# Autodesk Inventor assembly: 043.5-DQ(F,D-166-3)
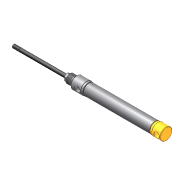
[picture p0: Inventor's stored thumbnail of the model, 180x180]
Saved by Autodesk Inventor 2012 (Build 160160000, 160)
## iProperties
Category: PARTsolutions
Created: 2013-01-20
Part Number: 043.5-DQ(F,D-166-3)
Catalog Web Link: www.cadenas.de
Description: Original Line Standard Air Cylinders -
Document SubType Name: Assembly
Designer: PARTsolutions
Mass: 32.8083 g
Surface Area: 278.831 cm^2
Volume: 32.8083 cm^3
Density: 1 g/cm^3
NB: 043.5-DQ(F,D-166-3)
NN: Original Line Standard Air Cylinders
NBSYN: $PNC.
LINA: 043.5-DQ
PSOL_MULTISOLIDPART: 0.0
PN: 043.5-DQ
PNC: 043.5-DQ(F,D-166-3)
PNA: (D-166-3)
DASH: -
BORE1: 0.75000000
BORE: 3/4" (04)
BOREPN: 04
STROKE: 3.500
STROKEALG: [0.011:50/0.001]
STROKE1: 3.500
ACTING: D
ACTINGALG: '' , 'Single Acting (SA)' , 'R' , 'Reverse Single Acting (SA)' , 'D' , 'Double Acting (SA)'
ACTINGPN: D
MNTALG: '' , 'Front Nose Mounting (SA)' , 'P' , 'Rear Pivot Mounting (SA)' , 'XP' , 'Double End or Pivot Mounting (SA)' , 'X' , 'Double End Mounting (SA)' , 'BF' , 'Front Block Mounting (SA)' , 'BR' , 'Rear Block Mounting for Vertical Positioning (SA)' , 'BFT' , 'Front Block Trunnion Mounting (SA)' , 'BRT' , 'Rear Block Trunnion Mounting (SA)'
DERALG: '' , 'N/A'
NRALG: '' , 'N/A'
BMALG: '' , 'N/A'
COALG: '' , 'N/A'
OOALG: '', 'N/A'
VO: Z
VOALG: 'Z' , 'N/A'
MALG: '', 'Without Magnet', 'M', 'With Magnet'
EEL: 0.000
EEMAX: 46.5000
EEALG: '', 'Without Extra Extension', 'EE', 'With Extra Extension'
EELALG: 0
EEPN1: 0.000
KALG: '' , 'N/A'
Q: Q
QALG: '' , 'Standard Port' , 'Q' , 'Side Port'
QPN: Q
YALG: '' , 'N/A'
FALG: '', 'Non-Coated (Standard)', 'F', 'Molycoated'
TALG: '' , 'Standard -20° to 200°F (-29° to 95°C)' , 'N' , 'Low Temperature' , 'V' , 'High Temperature'
BALG: '', 'W/out Bumpers' , 'B' , 'W/ Bumpers'
HALG: '', 'N/A'
SERALG: '' , 'Without Spring Extend/Return' , 'JS' , 'With Spring Return' , 'JR' , 'With Spring Extend'
SR: C
SRALG: 'C' , 'Standard Blackened Carbon Steel' , 'SR' , 'Stainless Steel [SR]'
SRCON: 1
WALG: '' , 'Without Wiper' , 'W' , 'With Wiper'
EALG: '' , 'Standard Seals/Lube' , 'E' , 'Non-Lube Seals/Lube'
HLALG: '' , 'Without Low Pressure Hydraulic' , 'HL' , 'With Low Pressure Hydraulic'
STALG: '' , 'N/A'
STPT1ALG: '' , 'N/A'
STPT2ALG: '' , 'N/A'
STPT3ALG: '' , 'N/A'
STPT4ALG: '' , 'N/A'
MBALG: '' , 'Without Mounting Bracket' , 'F,D-129' , 'D-129 (front)'
MBPNALL: D-129
PBALG: '' , 'N/A'
PRC: F,D-166-3
PRCALG: '' , 'W/out Pivot Rod Clevis' , 'F,D-166-3' , 'D-166-3 (front)'
PRCPN: (F,D-166-3)
PRCPNALL: D-166-3
TBALG: '' , 'N/A'
MNALG: '' , 'N/A'
TLEN: 4.7565
FRAC: 16.4700
RGDACCON: R
RHCON1: P
RHCONON: 1
FNUTCON: 1
RNUTCON: 0
FNUTPN: D-9
FNUTTRANS: 0.0000
RNUTTRANS: 0.0000
VHOLECON: 0
A1: 1.5940
A1N: 0.8750
A1P: 1.5940
A1B: 1.5940
A4: 0.2525
A4N: 0.3130
A4P: 0.2525
A5: 0.0300
A1H: 0.531
A1NH: 0.5310
A1PH: 1.5940
A1BH: 1.0940
A1SH: 1.2190
A2H: 0.2190
A2NH: 0.2190
LENGTH: 2.9700
LENGTH1: 2.9700
LENGTH2: 3.0300
MUL: 3.5000
MUL11: 3.5000
MUL22: 9.415
MUL33: 5.9150
MUL2: 3.5000
MUL211: 3.5000
MUL222: 2.6900
MUL233: 1.6900
SSS: 7.0000
RGLEN: 1.3715
RHLEN: 0.3420
SSS1: 4.0000
A13: 1.3120
DIF: 0.0000
G5: 0.6250
ON: 0
SSADD: 0.0000
BADD: 0.0000
MADD: 0.0000
NVADD: 0.0000
TRACKL: 4.4665
TRACKCON: D-74168
TRIMCON: 0
TRIMCON1: 0
FSPACE: 0.7247
SPACE: 0.0804
TEXT: 0.1406
S1: 1.0000
D1: 0.8325
D1N: 0.8050
D1B: 0.8625
D1P: 0.8325
FA: 0.940
RA: 0.9400
PPATH: standard_air_cylinder_asmtpl.prj
MATALGHTML: <b>Standard Original Line:</b><dl><dt>Rod:</dt><dd>- Stainless Steel</dd><dd>&nbsp;&nbsp;(5/16 ? 9/16 Bores)</dd><dd>- High Strength Carbon Steel</dd><dd>&nbsp;&nbsp;(3/4 ? 3 Bore)</dd><dd>- Stainless Steel</dd><dd>&nbsp;&nbsp;(?X? style DXP/DX/DXDE?)</dd><dt>Bearings:</dt><dd>- Sintered Bronze</dd><dt>Body:</dt><dd>- 304 Stainless Steel</dd><dt>End Caps:</dt><dd>- Aluminum</dd><dt>Seals:</dt><dd>- Buna N</dd></dl>
ASSCFGPRA: 04D
PRCPNA: (D-166-3)
ASSOPTACC: STPT4
A: 6.91
HADD: 0.0000
WFL: 0.250
QADD: 0.440
QADD1: 0.440
TEST: 3.0000
STDNUTF: 1
STDNUTR: 0
KT: DUMMY
CreationOption_UseAsmMates: false
SUPPLIER: Bimba
ARTICLENO: 043.5-DQ(F,D-166-3)
BOMINFO: 043.5-DQ
CREATOR: CADENAS GmbH
PSOL_IDENT_0: {\\10.0.0.242\data_v9\23d-libs\bimba\bimba\bimba_imperial\bimba_full_line\original_line_cylinders\st
PSOL_IDENT_1: andard_air_cylinders\standard_air_cylinder_asmtab.prj},318 {VTYP=3D},{STYP=ASSTAB},{NB=043.5-DQ(F,D-
PSOL_IDENT_2: 166-3)},{LINA=043.5-DQ},{NN=Original Line Standard Air Cylinders},{DATE=06.09.2012 11:26:56},{GEOMDA
PSOL_IDENT_3: TE=06.09.2012},{VERSION=},{LINEID=50},{LINESUBID=-1},{WBVAR=STROKE,ACTING,MNT,DER,NR,BM,CO,OO,VO,M,E
PSOL_IDENT_4: E,EEL,K,Q,Y,G,T,B,H,SER,SR,NT,W,HL,STPT1,STPT2,STPT3,STPT4,MB,PB,PRC,TB,MN}  {NB=043.5-DQ(F,D-166-3)
PSOL_IDENT_5: },{LINA=043.5-DQ},{KT=DUMMY},{PN=043.5-DQ},{PNC=043.5-DQ(F,D-166-3)},{PNA=(D-166-3)},{DASH=-},{BORE1
PSOL_IDENT_6: =0.75000000},{BORE=3/4\" (04)},{BOREPN=04},{STROKE=3.500},{STROKEALG=[0.011:50/0.001]},{STROKE1=3.50
PSOL_IDENT_7: 0},{ACTING=D},{ACTINGALG= '' , 'Single Acting (SA)' , 'R' , 'Reverse Single Acting (SA)' , 'D' , 'Do
PSOL_IDENT_8: uble Acting (SA)' },{ACTINGPN=D},{MNT=},{MNTALG= '' , 'Front Nose Mounting (SA)' , 'P' , 'Rear Pivot
PSOL_IDENT_9: Mounting (SA)' , 'XP' , 'Double End or Pivot Mounting (SA)' , 'X' , 'Double End Mounting (SA)' , 'B
PSOL_IDENT_10: F' , 'Front Block Mounting (SA)' , 'BR' , 'Rear Block Mounting for Vertical Positioning (SA)' , 'BFT
PSOL_IDENT_11: ' , 'Front Block Trunnion Mounting (SA)' , 'BRT' , 'Rear Block Trunnion Mounting (SA)' },{TYPE=},{MN
PSOL_IDENT_12: TPN=},{DER=},{DERALG= '' , 'N/A' },{NR=},{NRALG= '' , 'N/A' },{NRPN=},{BM=},{BMALG= '' , 'N/A' },{BM
PSOL_IDENT_13: PN=},{CO=},{COALG= '' , 'N/A' },{OO=},{OOALG= '', 'N/A' },{OOPN=},{VO=Z},{VOALG= 'Z' , 'N/A' },{VOPN
PSOL_IDENT_14: =},{OOVOPN=},{M=},{MALG= '', 'Without Magnet', 'M', 'With Magnet' },{EE=},{EEL=0.000},{EEMAX=46.5000
PSOL_IDENT_15: },{EEALG= '', 'Without Extra Extension', 'EE', 'With Extra Extension' },{EELALG=0},{EEPN=},{EEPN1=0.
PSOL_IDENT_16: 000},{K=},{KALG= '' , 'N/A' },{KPN=},{Q=Q},{QALG= '' , 'Standard Port' , 'Q' , 'Side Port' },{QPN=Q}
PSOL_IDENT_17: ,{Y=},{YALG= '' , 'N/A' },{YPN=},{YCON=},{F=},{FALG= '', 'Non-Coated (Standard)', 'F', 'Molycoated'
PSOL_IDENT_18: },{FPN=},{G=},{GPN=},{GPN99=},{T=},{TALG= '' , 'Standard -20° to 200°F (-29° to 95°C)' , 'N' , 'Low
PSOL_IDENT_19: Temperature' , 'V' , 'High Temperature' },{NPN=},{VPN=},{B=},{BALG= '', 'W/out Bumpers' , 'B' , 'W/
PSOL_IDENT_20: Bumpers' },{BPN=},{H=},{HALG= '', 'N/A' },{HPN=},{SER=},{SERALG= '' , 'Without Spring Extend/Return'
PSOL_IDENT_21: , 'JS' , 'With Spring Return' , 'JR' , 'With Spring Extend' },{SR=C},{SRALG= 'C' , 'Standard Blacke
PSOL_IDENT_22: ned Carbon Steel' , 'SR' , 'Stainless Steel [SR]' },{SRPN=},{SRCON=1},{NT=},{NTPN=},{W=},{WALG= '' ,
PSOL_IDENT_23: 'Without Wiper' , 'W' , 'With Wiper' },{WPN=},{E=},{EALG= '' , 'Standard Seals/Lube' , 'E' , 'Non-L
PSOL_IDENT_24: ube Seals/Lube' },{EPN=},{HL=},{HLALG= '' , 'Without Low Pressure Hydraulic' , 'HL' , 'With Low Pres
PSOL_IDENT_25: sure Hydraulic' },{ST=},{STALG= '' , 'N/A' },{STPT1=},{STPT1ALG= '' , 'N/A' },{STPT2=},{STPT2ALG= ''
PSOL_IDENT_26: , 'N/A' },{STPT3=},{STPT3ALG= '' , 'N/A' },{STPT4=},{STPT4ALG= '' , 'N/A' },{STPN=},{MB=},{MBALG= '
PSOL_IDENT_27: ' , 'Without Mounting Bracket' , 'F,D-129' , 'D-129 (front)' },{MBPN=},{MBPNALL=D-129},{MBPNALLREAR=
PSOL_IDENT_28: },{PB=},{PBALG= '' , 'N/A' },{PBPN=},{PBPNALL=},{PRC=F,D-166-3},{PRCALG= '' , 'W/out Pivot Rod Clevi
PSOL_IDENT_29: s' , 'F,D-166-3' , 'D-166-3 (front)' },{PRCPN=(F,D-166-3)},{PRCPNALL=D-166-3},{TB=},{TBALG= '' , 'N/
PSOL_IDENT_30: A' },{TBPN=},{TBPNALL=},{MN=},{MNALG= '' , 'N/A' },{MNPN=},{MNCONF=},{MNCONR=},{TLEN=4.7565},{FRAC=1
PSOL_IDENT_31: 6.4700},{RGCON=},{RGDACCON=R},{RHCON=},{RHCON1=P},{RHCONON=1},{RHACCON=},{FNUTCON=1},{RNUTCON=0},{FN
PSOL_IDENT_32: UTPN=D-9},{RNUTPN=},{FNUTTRANS=0.0000},{RNUTTRANS=0.0000},{VHOLECON=0},{A1=1.5940},{A1N=0.8750},{A1P
PSOL_IDENT_33: =1.5940},{A1B=1.5940},{A4=0.2525},{A4N=0.3130},{A4P=0.2525},{A5=0.0300},{A1H=0.531},{A1NH=0.5310},{A
PSOL_IDENT_34: 1PH=1.5940},{A1BH=1.0940},{A1SH=1.2190},{A2H=0.2190},{A2NH=0.2190},{LENGTH=2.9700},{LENGTH1=2.9700},
PSOL_IDENT_35: {LENGTH2=3.0300},{MUL=3.5000},{MUL11=3.5000},{MUL22=9.415},{MUL33=5.9150},{MUL2=3.5000},{MUL211=3.50
PSOL_IDENT_36: 00},{MUL222=2.6900},{MUL233=1.6900},{SSS=7.0000},{RGLEN=1.3715},{RHLEN=0.3420},{SSS1=4.0000},{A13=1.
PSOL_IDENT_37: 3120},{DIF=0.0000},{G5=0.6250},{ON=0},{SSADD=0.0000},{BADD=0.0000},{MADD=0.0000},{NVADD=0.0000},{TRA
PSOL_IDENT_38: CKL=4.4665},{TRACKCON=D-74168},{TRIMCON=0},{TRIMCON1=0},{PINCON=},{FSPACE=0.7247},{SPACE=0.0804},{TE
PSOL_IDENT_39: XT=0.1406},{S1=1.0000},{D1=0.8325},{D1N=0.8050},{D1B=0.8625},{D1P=0.8325},{FA=0.940},{RA=0.9400},{PP
PSOL_IDENT_40: ATH=standard_air_cylinder_asmtpl.prj},{MATALGHTML=<b>Standard Original Line:</b><dl><dt>Rod:</dt><dd
PSOL_IDENT_41: >- Stainless Steel</dd><dd>&nbsp;&nbsp;(5/16 ? 9/16 Bores)</dd><dd>- High Strength Carbon Steel</dd>
PSOL_IDENT_42: <dd>&nbsp;&nbsp;(3/4 ? 3 Bore)</dd><dd>- Stainless Steel</dd><dd>&nbsp;&nbsp;(?X? style DXP/DX/DXDE?
PSOL_IDENT_43: )</dd><dt>Bearings:</dt><dd>- Sintered Bronze</dd><dt>Body:</dt><dd>- 304 Stainless Steel</dd><dt>En
PSOL_IDENT_44: d Caps:</dt><dd>- Aluminum</dd><dt>Seals:</dt><dd>- Buna N</dd></dl>},{ASSCFGPRA=04D},{MBPNA=},{MNPN
PSOL_IDENT_45: A=},{PRCPNA=(D-166-3)},{ASSOPTACC=STPT4},{A=6.91},{HADD=0.0000},{WFL=0.25},{QADD=0.440},{QADD1=0.440
PSOL_IDENT_46: },{TEST=3.0000},{MNTB=},{STDNUTF=1},{STDNUTR=0}
Title: 043.5-DQ
Author: Cadenas PARTsolutions
## Documents named in this file (7)
- Z:\UserData\Documents\Inventor\team1885frc\Pneumatics\043-5_DQ_3-5inStrokex075\043_5_DQ_F_D_166_3_.iam
- Z:\UserData\Documents\Inventor\team1885frc\Pneumatics\043-5_DQ_3-5inStrokex075\04RQ000_rod_guide.ipt
- Z:\UserData\Documents\Inventor\team1885frc\Pneumatics\043-5_DQ_3-5inStrokex075\043_5_DQ0_rod.ipt
- Z:\UserData\Documents\Inventor\team1885frc\Pneumatics\043-5_DQ_3-5inStrokex075\D_166_3_dummy.ipt
- Z:\UserData\Documents\Inventor\team1885frc\Pneumatics\043-5_DQ_3-5inStrokex075\D_344.ipt
- Z:\UserData\Documents\Inventor\team1885frc\Pneumatics\043-5_DQ_3-5inStrokex075\04R_4_75650C.ipt
- Z:\UserData\Documents\Inventor\team1885frc\Pneumatics\043-5_DQ_3-5inStrokex075\04PQ0000_rear_head.ipt
## Components (6 placed, 6 different names)
1. 04RQ000_rod_guide:1 — Mate:1
2. D-166-3-dummy:1
3. D-344:1
4. 04R-4.75650C:1
5. 04PQ0000_rear_head:1 — Mate:2
6. 043.5-DQ0_rod:1 — Mate:1, Mate:2
## Relationships (2: Mate 2)
- Mate:1: 04RQ000_rod_guide:1 ↔ 043.5-DQ0_rod:1
- Mate:2: 04PQ0000_rear_head:1 ↔ 043.5-DQ0_rod:1
